# Autodesk Inventor assembly: AXp2c
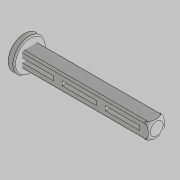
[picture p0: Inventor's stored thumbnail of the model, 180x180]
Saved by Autodesk Inventor 2020 (Build 240168000, 168)
## iProperties
Created: 2019-05-09
Part Number: AXp2c
Document SubType Name: Assembly
Designer: Varga Daniel
Author: Varga Daniel
## Documents named in this file (4)
- C:\!_Dani\!_cloud\OneDrive\!_munka\Revolution\StructuralParts\Axles\AXpXc\AXp3c.iam
- C:\!_Dani\!_cloud\OneDrive\!_munka\Revolution\StructuralParts\Axles\Axle_collar.ipt
- C:\!_Dani\!_cloud\OneDrive\!_munka\Revolution\StructuralParts\Axles\One_sided_axle_base.ipt
- C:\!_Dani\!_cloud\OneDrive\!_munka\Revolution\StructuralParts\Axles\One_sided_axle_base\One_sided_axle_base-30.ipt
## Components (2 placed, 2 different names)
1. Axle_collar:1 — Mate:2, Mate:3, Flush:1
2. One_sided_axle_base-30:1 — Mate:4, Mate:5, Mate:6
## Relationships (6: Mate 5, Flush 1)
- Mate:2: Axle_collar:1
- Mate:3: Axle_collar:1
- Flush:1: Axle_collar:1
- Mate:4: One_sided_axle_base-30:1
- Mate:5: One_sided_axle_base-30:1
- Mate:6: One_sided_axle_base-30:1
